# Autodesk Inventor assembly: ASDSAssemblyREV3
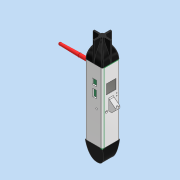
[picture p0: Inventor's stored thumbnail of the model, 180x180]
Saved by Autodesk Inventor 2020.3 (Build 243373000, 373)
## iProperties
Created: 2020-06-02
Part Number: ASDSAssemblyREV3
Document SubType Name: Assembly
Designer: Derek Wider
Author: Derek Wider
## Documents named in this file (8)
- D:\Documents\GitHub\Submarine-project\CAD\ASDS\REV3\ASDSAssemblyREV3.iam
- D:\Documents\GitHub\Submarine-project\CAD\ASDS\REV3\Hull_REV3.ipt
- D:\Documents\GitHub\Submarine-project\CAD\common\VideoTransmitter.ipt
- D:\Documents\GitHub\Submarine-project\CAD\ASDS\ASDSBattery.ipt
- D:\Documents\GitHub\Submarine-project\CAD\ASDS\Antenna.ipt
- D:\Documents\GitHub\Submarine-project\CAD\ASDS\REV3\arduino_radio_volume.ipt
- D:\Documents\GitHub\Submarine-project\CAD\ASDS\Aft.ipt
- D:\Documents\GitHub\Submarine-project\CAD\ASDS\Fore.ipt
## Components (7 placed, 7 different names)
1. Hull_REV3:1 — Mate:1, Mate:2, Mate:4, Mate:5, Mate:6, Mate:7, Mate:8, Flush:1, Mate:9, Mate:10, Mate:11, Mate:12, Mate:13, Mate:14
2. VideoTransmitter:1 — Mate:4, Mate:5, Mate:6
3. ASDSBattery:1 — Mate:1, Mate:2
4. Antenna:1 — Mate:8, Flush:1
5. arduino_radio_volume:1 — Mate:7
6. Aft:1 — Mate:9, Mate:10, Mate:11
7. Fore:1 — Mate:12, Mate:13, Mate:14
## Relationships (14: Mate 13, Flush 1)
- Mate:1: Hull_REV3:1 ↔ ASDSBattery:1
- Mate:2 (5.08 mm): Hull_REV3:1 ↔ ASDSBattery:1
- Mate:4: Hull_REV3:1 ↔ VideoTransmitter:1
- Mate:5 (0.508 mm): Hull_REV3:1 ↔ VideoTransmitter:1
- Mate:6 (0.508 mm): Hull_REV3:1 ↔ VideoTransmitter:1
- Mate:7: Hull_REV3:1 ↔ arduino_radio_volume:1
- Mate:8: Hull_REV3:1 ↔ Antenna:1
- Flush:1: Hull_REV3:1 ↔ Antenna:1
- Mate:9: Hull_REV3:1 ↔ Aft:1
- Mate:10: Hull_REV3:1 ↔ Aft:1
- Mate:11: Hull_REV3:1 ↔ Aft:1
- Mate:12: Hull_REV3:1 ↔ Fore:1
- Mate:13: Hull_REV3:1 ↔ Fore:1
- Mate:14: Hull_REV3:1 ↔ Fore:1
